# Autodesk Inventor assembly: base_link
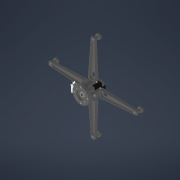
[picture p0: Inventor's stored thumbnail of the model, 180x180]
Saved by Autodesk Inventor 2022 (Build 260153070, 153G)
## iProperties
Created: 2021-11-20
Part Number: base_link
Document SubType Name: Assembly
Designer: Teo
Title: Predstavitev sklopa
Author: Teo
## Documents named in this file (15)
- D:\Zaključna\Roka\Priloge\IPT_files\Assemblies\base_link.iam
- D:\Zaključna\Roka\Priloge\IPT_files\Stepper_nema17.ipt
- D:\Zaključna\Roka\Priloge\IPT_files\Assemblies\reductor.iam
- D:\Zaključna\Roka\Priloge\IPT_files\Stator_lite.ipt
- D:\Zaključna\Roka\Priloge\IPT_files\Base_lite.ipt
- D:\Zaključna\Roka\Priloge\IPT_files\Leg_lite.ipt
- D:\Zaključna\Roka\Priloge\IPT_files\Foot_lite.ipt
- C:\Users\Teo\Documents\Inventor\Content Center Files\R2022\en-US\DIN 912\DIN 912 - M5 x 0.8 x 35 x 22.ipt
- C:\Users\Teo\Documents\Inventor\Content Center Files\R2022\en-US\DIN 912\DIN 912 - M3 x 0.5 x 25 x 18.ipt
- C:\Users\Teo\Documents\Inventor\Content Center Files\R2022\en-US\DIN 439-2\DIN 439 - M5 x 0.8.ipt
- C:\Users\Teo\Documents\Inventor\Content Center Files\R2022\en-US\DIN 912\DIN 912 - M3 x 0.5 x 30 x 18.ipt
- C:\Users\Teo\Documents\Inventor\Content Center Files\R2022\en-US\DIN 439-2\DIN 439 - M3 x 0.5.ipt
- C:\Users\Teo\Documents\Inventor\Content Center Files\R2022\en-US\DIN 912\DIN 912 - M5 x 0.8 x 20 x 18.ipt
- D:\Zaključna\Roka\Priloge\IPT_files\Limit_switch.ipt
- C:\Users\Teo\Documents\Inventor\Content Center Files\R2022\en-US\DIN 912\DIN 912 - M3 x 0.5 x 16 x 14.75.ipt
## Components (39 placed, 14 different names)
1. Stepper_nema17:1 — Mate:1, Mate:2, Mate:3, Mate:4
2. reductor:1 [sub-assembly] — Mate:1, Mate:2, Mate:3, Mate:4, Mate:5, Mate:6, Mate:7
3. Stator_lite:1 — Mate:5, Mate:6, Mate:7, Mate:8, Mate:9, Mate:10, Mate:27, Mate:28, Mate:29, Mate:30, Mate:31, Mate:32, Mate:33, Mate:34, Mate:35, Mate:37, Mate:39, Mate:41, Mate:52, Mate:54, Mate:56, Mate:58, Mate:59, Mate:60, Mate:61, Mate:62
4. Base_lite:1 — Mate:8, Mate:9, Mate:10, Mate:11, Mate:12, Angle:1, Mate:13, Mate:14, Angle:2, Mate:15, Mate:16, Angle:3, Mate:17, Mate:18, Angle:4, Mate:36, Mate:38, Mate:40, Mate:42, Mate:43, Mate:44, Mate:45, Mate:46, Mate:47, Mate:48, Mate:49, Mate:50, Mate:64, Mate:66, Mate:68, Mate:70, Mate:79, Mate:80, Angle:5
5. Leg_lite:1 — Mate:11, Mate:12, Angle:1, Mate:19, Mate:20, Mate:73
6. Leg_lite:2 — Mate:13, Mate:14, Angle:2, Mate:21, Mate:22, Mate:71
7. Leg_lite:3 — Mate:15, Mate:16, Angle:3, Mate:23, Mate:24, Mate:75
8. Leg_lite:4 — Mate:17, Mate:18, Angle:4, Mate:25, Mate:26, Mate:77
9. Foot_lite:1 — Mate:19, Mate:20, Mate:74
10. Foot_lite:2 — Mate:21, Mate:22, Mate:72
11. Foot_lite:3 — Mate:23, Mate:24, Mate:76
12. Foot_lite:4 — Mate:25, Mate:26, Mate:78
13. Limit_switch:1 — Mate:79, Mate:80, Angle:5, Mate:81, Mate:82, Mate:83, Mate:84
14. DIN 912 - replaced by DIN EN ISO 4762 M3 x 30:4 — Mate:27, Mate:28
15. DIN 912 - replaced by DIN EN ISO 4762 M3 x 30:2 — Mate:29, Mate:30
16. DIN 912 - replaced by DIN EN ISO 4762 M3 x 30:1 — Mate:31, Mate:32
17. DIN 912 - replaced by DIN EN ISO 4762 M3 x 30:3 — Mate:33, Mate:34
18. DIN 912 - replaced by DIN EN ISO 4762 M5 x 35:2 — Mate:35, Mate:36, Mate:55
19. DIN 912 - replaced by DIN EN ISO 4762 M5 x 35:1 — Mate:37, Mate:38, Mate:53
20. DIN 912 - replaced by DIN EN ISO 4762 M5 x 35:3 — Mate:39, Mate:40, Mate:57
21. DIN 912 - replaced by DIN EN ISO 4762 M5 x 35:4 — Mate:41, Mate:42, Mate:51
22. DIN 912 - replaced by DIN EN ISO 4762 M3 x 25:2 — Mate:43, Mate:44, Mate:67
23. DIN 912 - replaced by DIN EN ISO 4762 M3 x 25:4 — Mate:45, Mate:46, Mate:63
24. DIN 912 - replaced by DIN EN ISO 4762 M3 x 25:1 — Mate:47, Mate:48, Mate:69
25. DIN 912 - replaced by DIN EN ISO 4762 M3 x 25:3 — Mate:49, Mate:50, Mate:65
26. DIN 912 - replaced by DIN EN ISO 4762 M5 x 20:1 — Mate:71, Mate:72
27. DIN 912 - replaced by DIN EN ISO 4762 M5 x 20:2 — Mate:73, Mate:74
28. DIN 912 - replaced by DIN EN ISO 4762 M5 x 20:3 — Mate:75, Mate:76
29. DIN 912 - replaced by DIN EN ISO 4762 M5 x 20:4 — Mate:77, Mate:78
30. DIN 439-2 - replaced by DIN EN 24035/28675 M5:1 — Mate:51, Mate:52, Mate:60
31. DIN 439-2 - replaced by DIN EN 24035/28675 M5:2 — Mate:53, Mate:54, Mate:61
32. DIN 439-2 - replaced by DIN EN 24035/28675 M5:3 — Mate:55, Mate:56, Mate:62
33. DIN 439-2 - replaced by DIN EN 24035/28675 M5:4 — Mate:57, Mate:58, Mate:59
34. DIN 439-2 - replaced by DIN EN 24035/28675 M3:1 — Mate:63, Mate:64
35. DIN 439-2 - replaced by DIN EN 24035/28675 M3:2 — Mate:65, Mate:66
36. DIN 439-2 - replaced by DIN EN 24035/28675 M3:3 — Mate:67, Mate:68
37. DIN 439-2 - replaced by DIN EN 24035/28675 M3:4 — Mate:69, Mate:70
38. DIN 912 - replaced by DIN EN ISO 4762 M3 x 16:1 — Mate:81, Mate:82
39. DIN 912 - replaced by DIN EN ISO 4762 M3 x 16:2 — Mate:83, Mate:84
## Relationships (89: Mate 84, Angle 5)
- Mate:1: Stepper_nema17:1 ↔ reductor:1
- Mate:2: Stepper_nema17:1 ↔ reductor:1
- Mate:3: Stepper_nema17:1 ↔ reductor:1
- Mate:4: Stepper_nema17:1 ↔ reductor:1
- Mate:5: reductor:1 ↔ Stator_lite:1
- Mate:6: reductor:1 ↔ Stator_lite:1
- Mate:7: reductor:1 ↔ Stator_lite:1
- Mate:8: Stator_lite:1 ↔ Base_lite:1
- Mate:9: Stator_lite:1 ↔ Base_lite:1
- Mate:10: Stator_lite:1 ↔ Base_lite:1
- Mate:11: Base_lite:1 ↔ Leg_lite:1
- Mate:12: Base_lite:1 ↔ Leg_lite:1
- Angle:1 (0 deg): Base_lite:1 ↔ Leg_lite:1
- Mate:13: Base_lite:1 ↔ Leg_lite:2
- Mate:14: Base_lite:1 ↔ Leg_lite:2
- Angle:2 (0 deg): Base_lite:1 ↔ Leg_lite:2
- Mate:15: Base_lite:1 ↔ Leg_lite:3
- Mate:16: Base_lite:1 ↔ Leg_lite:3
- Angle:3 (0 deg): Base_lite:1 ↔ Leg_lite:3
- Mate:17: Base_lite:1 ↔ Leg_lite:4
- Mate:18: Base_lite:1 ↔ Leg_lite:4
- Angle:4 (0 deg): Base_lite:1 ↔ Leg_lite:4
- Mate:19: Leg_lite:1 ↔ Foot_lite:1
- Mate:20: Leg_lite:1 ↔ Foot_lite:1
- Mate:21: Leg_lite:2 ↔ Foot_lite:2
- Mate:22: Leg_lite:2 ↔ Foot_lite:2
- Mate:23: Leg_lite:3 ↔ Foot_lite:3
- Mate:24: Leg_lite:3 ↔ Foot_lite:3
- Mate:25: Leg_lite:4 ↔ Foot_lite:4
- Mate:26: Leg_lite:4 ↔ Foot_lite:4
- Mate:27: Stator_lite:1 ↔ DIN 912 - replaced by DIN EN ISO 4762 M3 x 30:4
- Mate:28: Stator_lite:1 ↔ DIN 912 - replaced by DIN EN ISO 4762 M3 x 30:4
- Mate:29: Stator_lite:1 ↔ DIN 912 - replaced by DIN EN ISO 4762 M3 x 30:2
- Mate:30: Stator_lite:1 ↔ DIN 912 - replaced by DIN EN ISO 4762 M3 x 30:2
- Mate:31: Stator_lite:1 ↔ DIN 912 - replaced by DIN EN ISO 4762 M3 x 30:1
- Mate:32: Stator_lite:1 ↔ DIN 912 - replaced by DIN EN ISO 4762 M3 x 30:1
- Mate:33: Stator_lite:1 ↔ DIN 912 - replaced by DIN EN ISO 4762 M3 x 30:3
- Mate:34: Stator_lite:1 ↔ DIN 912 - replaced by DIN EN ISO 4762 M3 x 30:3
- Mate:35: Stator_lite:1 ↔ DIN 912 - replaced by DIN EN ISO 4762 M5 x 35:2
- Mate:36: Base_lite:1 ↔ DIN 912 - replaced by DIN EN ISO 4762 M5 x 35:2
- Mate:37: Stator_lite:1 ↔ DIN 912 - replaced by DIN EN ISO 4762 M5 x 35:1
- Mate:38: Base_lite:1 ↔ DIN 912 - replaced by DIN EN ISO 4762 M5 x 35:1
- Mate:39: Stator_lite:1 ↔ DIN 912 - replaced by DIN EN ISO 4762 M5 x 35:3
- Mate:40: Base_lite:1 ↔ DIN 912 - replaced by DIN EN ISO 4762 M5 x 35:3
- Mate:41: Stator_lite:1 ↔ DIN 912 - replaced by DIN EN ISO 4762 M5 x 35:4
- Mate:42: Base_lite:1 ↔ DIN 912 - replaced by DIN EN ISO 4762 M5 x 35:4
- Mate:43: Base_lite:1 ↔ DIN 912 - replaced by DIN EN ISO 4762 M3 x 25:2
- Mate:44: Base_lite:1 ↔ DIN 912 - replaced by DIN EN ISO 4762 M3 x 25:2
- Mate:45: Base_lite:1 ↔ DIN 912 - replaced by DIN EN ISO 4762 M3 x 25:4
- Mate:46: Base_lite:1 ↔ DIN 912 - replaced by DIN EN ISO 4762 M3 x 25:4
- Mate:47: Base_lite:1 ↔ DIN 912 - replaced by DIN EN ISO 4762 M3 x 25:1
- Mate:48: Base_lite:1 ↔ DIN 912 - replaced by DIN EN ISO 4762 M3 x 25:1
- Mate:49: Base_lite:1 ↔ DIN 912 - replaced by DIN EN ISO 4762 M3 x 25:3
- Mate:50: Base_lite:1 ↔ DIN 912 - replaced by DIN EN ISO 4762 M3 x 25:3
- Mate:51: DIN 912 - replaced by DIN EN ISO 4762 M5 x 35:4 ↔ DIN 439-2 - replaced by DIN EN 24035/28675 M5:1
- Mate:52: Stator_lite:1 ↔ DIN 439-2 - replaced by DIN EN 24035/28675 M5:1
- Mate:53: DIN 912 - replaced by DIN EN ISO 4762 M5 x 35:1 ↔ DIN 439-2 - replaced by DIN EN 24035/28675 M5:2
- Mate:54: Stator_lite:1 ↔ DIN 439-2 - replaced by DIN EN 24035/28675 M5:2
- Mate:55: DIN 912 - replaced by DIN EN ISO 4762 M5 x 35:2 ↔ DIN 439-2 - replaced by DIN EN 24035/28675 M5:3
- Mate:56: Stator_lite:1 ↔ DIN 439-2 - replaced by DIN EN 24035/28675 M5:3
- Mate:57: DIN 912 - replaced by DIN EN ISO 4762 M5 x 35:3 ↔ DIN 439-2 - replaced by DIN EN 24035/28675 M5:4
- Mate:58: Stator_lite:1 ↔ DIN 439-2 - replaced by DIN EN 24035/28675 M5:4
- Mate:59: Stator_lite:1 ↔ DIN 439-2 - replaced by DIN EN 24035/28675 M5:4
- Mate:60: Stator_lite:1 ↔ DIN 439-2 - replaced by DIN EN 24035/28675 M5:1
- Mate:61: Stator_lite:1 ↔ DIN 439-2 - replaced by DIN EN 24035/28675 M5:2
- Mate:62: Stator_lite:1 ↔ DIN 439-2 - replaced by DIN EN 24035/28675 M5:3
- Mate:63: DIN 912 - replaced by DIN EN ISO 4762 M3 x 25:4 ↔ DIN 439-2 - replaced by DIN EN 24035/28675 M3:1
- Mate:64: Base_lite:1 ↔ DIN 439-2 - replaced by DIN EN 24035/28675 M3:1
- Mate:65: DIN 912 - replaced by DIN EN ISO 4762 M3 x 25:3 ↔ DIN 439-2 - replaced by DIN EN 24035/28675 M3:2
- Mate:66: Base_lite:1 ↔ DIN 439-2 - replaced by DIN EN 24035/28675 M3:2
- Mate:67: DIN 912 - replaced by DIN EN ISO 4762 M3 x 25:2 ↔ DIN 439-2 - replaced by DIN EN 24035/28675 M3:3
- Mate:68: Base_lite:1 ↔ DIN 439-2 - replaced by DIN EN 24035/28675 M3:3
- Mate:69: DIN 912 - replaced by DIN EN ISO 4762 M3 x 25:1 ↔ DIN 439-2 - replaced by DIN EN 24035/28675 M3:4
- Mate:70: Base_lite:1 ↔ DIN 439-2 - replaced by DIN EN 24035/28675 M3:4
- Mate:71: Leg_lite:2 ↔ DIN 912 - replaced by DIN EN ISO 4762 M5 x 20:1
- Mate:72: Foot_lite:2 ↔ DIN 912 - replaced by DIN EN ISO 4762 M5 x 20:1
- Mate:73: Leg_lite:1 ↔ DIN 912 - replaced by DIN EN ISO 4762 M5 x 20:2
- Mate:74: Foot_lite:1 ↔ DIN 912 - replaced by DIN EN ISO 4762 M5 x 20:2
- Mate:75: Leg_lite:3 ↔ DIN 912 - replaced by DIN EN ISO 4762 M5 x 20:3
- Mate:76: Foot_lite:3 ↔ DIN 912 - replaced by DIN EN ISO 4762 M5 x 20:3
- Mate:77: Leg_lite:4 ↔ DIN 912 - replaced by DIN EN ISO 4762 M5 x 20:4
- Mate:78: Foot_lite:4 ↔ DIN 912 - replaced by DIN EN ISO 4762 M5 x 20:4
- Mate:79: Base_lite:1 ↔ Limit_switch:1
- Mate:80: Base_lite:1 ↔ Limit_switch:1
- Angle:5 (0 deg): Base_lite:1 ↔ Limit_switch:1
- Mate:81: Limit_switch:1 ↔ DIN 912 - replaced by DIN EN ISO 4762 M3 x 16:1
- Mate:82: Limit_switch:1 ↔ DIN 912 - replaced by DIN EN ISO 4762 M3 x 16:1
- Mate:83: Limit_switch:1 ↔ DIN 912 - replaced by DIN EN ISO 4762 M3 x 16:2
- Mate:84: Limit_switch:1 ↔ DIN 912 - replaced by DIN EN ISO 4762 M3 x 16:2
